# Autodesk Inventor assembly: 20170529set1_to_print
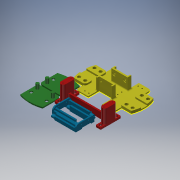
[picture p0: Inventor's stored thumbnail of the model, 180x180]
Saved by Autodesk Inventor 2017 SP1 (Build 210196100, 196)
## iProperties
Created: 2016-07-26
Part Number: 20170529set1_to_print
Material: Générique
Document SubType Name: Assembly
Designer: tmonglon
Author: tmonglon
## Documents named in this file (5)
- D:\Inventor\Ahmet\29_mai_2017\20170525_ebug_chassis\20170529_ebug_chassis\20170529set1_to_print.iam
- D:\Inventor\Ahmet\mai_2017\modified\green_part_modified.ipt
- D:\Inventor\Ahmet\mai_2017\modified\red_part_modified.ipt
- D:\Inventor\Ahmet\mai_2017\modified\blue_part_modified.ipt
- D:\Inventor\Ahmet\mai_2017\modified\yellow_part_modified.ipt
## Components (6 placed, 4 different names)
1. yellow_part_modified:1 — Affleurement:1, Placage:1, Affleurement:4, Placage:4
2. green_part_modified:1 — Affleurement:2, Placage:2, Affleurement:3, Placage:3
3. green_part_modified:2 — Affleurement:1, Affleurement:2, Placage:1, Placage:2, Affleurement:3
4. red_part_modified:1 — Affleurement:4, Placage:3, Placage:4, Affleurement:5, Placage:5, Placage:6
5. blue_part_modified:1 — Affleurement:5, Placage:5, Placage:6, Affleurement:6, Placage:7
6. blue_part_modified:2 — Affleurement:6, Placage:7
## Relationships (13: Mate 7, Flush 6)
- Affleurement:1 [Flush]: yellow_part_modified:1 ↔ green_part_modified:2
- Affleurement:2 [Flush]: green_part_modified:1 ↔ green_part_modified:2
- Placage:1 [Mate] (2 mm): yellow_part_modified:1 ↔ green_part_modified:2
- Placage:2 [Mate] (2 mm): green_part_modified:1 ↔ green_part_modified:2
- Affleurement:3 [Flush]: green_part_modified:1 ↔ green_part_modified:2
- Affleurement:4 [Flush]: yellow_part_modified:1 ↔ red_part_modified:1
- Placage:3 [Mate] (2 mm): green_part_modified:1 ↔ red_part_modified:1
- Placage:4 [Mate] (2 mm): yellow_part_modified:1 ↔ red_part_modified:1
- Affleurement:5 [Flush]: red_part_modified:1 ↔ blue_part_modified:1
- Placage:5 [Mate] (2 mm): red_part_modified:1 ↔ blue_part_modified:1
- Placage:6 [Mate] (5 mm): red_part_modified:1 ↔ blue_part_modified:1
- Affleurement:6 [Flush]: blue_part_modified:1 ↔ blue_part_modified:2
- Placage:7 [Mate] (2 mm): blue_part_modified:1 ↔ blue_part_modified:2
